# Autodesk Inventor assembly: Assembly3
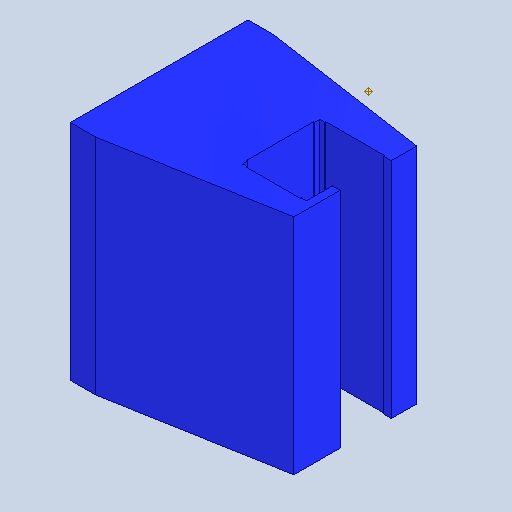
[picture p0: Inventor's stored thumbnail of the model, 512x512]
Saved by Autodesk Inventor 2022 (Build 260153000, 153)
## iProperties
Created: 2022-03-21
Part Number: Assembly3
Document SubType Name: Assembly
Designer: Nick
Author: Nick
## Documents named in this file (3)
- Y:\Projects\Bibble0\3D printed\Z Axis\Z Belt Housing HSI.iam
- Y:\Projects\Bibble0\3D printed\Z Axis\Z Belt Housing.ipt
- Y:\Projects\Bibble0\Hardware\M3 Heat Set Inserts.ipt
## Components (2 placed, 2 different names)
1. Z Belt Housing:1 — Insert:1
2. M3 Heat Set Inserts:1 — Insert:1
## Relationships (1: Insert 1)
- Insert:1: Z Belt Housing:1 ↔ M3 Heat Set Inserts:1
